# Autodesk Inventor assembly: 2016_IEEE_SouteastCon_Court
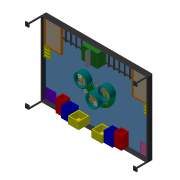
[picture p0: Inventor's stored thumbnail of the model, 180x180]
Saved by Autodesk Inventor 2015 (Build 190159000, 159)
## iProperties
Created: 2015-03-03
Part Number: 2016_IEEE_SouteastCon_Court
Document SubType Name: Assembly
Designer: Vukica
Author: Vukica
## Documents named in this file (16)
- C:\Users\Vukica\Dropbox\IEEE\hardware rules\2016Hardware_Court\2016_IEEE_SouteastCon_Court.iam
- C:\Users\Vukica\Dropbox\IEEE\hardware rules\2016Hardware_Court\Base.ipt
- C:\Users\Vukica\Dropbox\IEEE\hardware rules\2016Hardware_Court\Ship area.ipt
- C:\Users\Vukica\Dropbox\IEEE\hardware rules\2016Hardware_Court\Starting position pink.ipt
- C:\Users\Vukica\Dropbox\IEEE\hardware rules\2016Hardware_Court\Starting position purple.ipt
- C:\Users\Vukica\Dropbox\IEEE\hardware rules\2016Hardware_Court\Rail zone.ipt
- C:\Users\Vukica\Dropbox\IEEE\hardware rules\2016Hardware_Court\Beacon.ipt
- C:\Users\Vukica\Dropbox\IEEE\hardware rules\2016Hardware_Court\Side 84 in by 6 in by half inch.ipt
- C:\Users\Vukica\Dropbox\IEEE\hardware rules\2016Hardware_Court\Side 120 in by 6 in by half inch.ipt
- C:\Users\Vukica\Dropbox\IEEE\hardware rules\2016Hardware_Court\Hill.ipt
- C:\Users\Vukica\Dropbox\IEEE\hardware rules\2016Hardware_Court\Red truck.ipt
- C:\Users\Vukica\Dropbox\IEEE\hardware rules\2016Hardware_Court\Blue truck.ipt
- C:\Users\Vukica\Dropbox\IEEE\hardware rules\2016Hardware_Court\Yellow truck.ipt
- C:\Users\Vukica\Dropbox\IEEE\hardware rules\2016Hardware_Court\Island.ipt
- C:\Users\Vukica\Dropbox\IEEE\hardware rules\2016Hardware_Court\Gold bar.ipt
- C:\Users\Vukica\Dropbox\IEEE\hardware rules\2016Hardware_Court\White shipping good.ipt
## Components (43 placed, 15 different names)
1. Base:1 — Mate:1, Flush:1, Flush:2, Mate:2, Flush:3, Flush:4, Mate:3, Flush:5, Flush:6, Mate:4, Flush:7, Flush:8, Mate:5, Flush:9, Mate:7, Flush:11, Mate:9, Flush:12, Flush:13, Flush:15, Mate:10, Mate:11, Flush:16, Flush:18, Mate:12, Mate:17, Mate:20, Mate:22, Mate:25, Mate:28, Mate:30, Mate:33, Mate:36, Mate:38, Mate:40, Mate:43, Mate:46, Mate:53, Mate:55
2. Ship area:1 — Mate:1, Flush:1, Flush:2, Mate:6, Mate:49
3. Ship area:2 — Mate:2, Flush:3, Flush:4, Mate:8, Flush:10, Mate:54
4. Starting position pink:1 — Mate:4, Flush:7, Flush:8
5. Starting position purple:1 — Mate:3, Flush:5, Flush:6
6. Rail zone:1 — Mate:5, Mate:6, Flush:9
7. Rail zone:2 — Mate:7, Mate:8, Flush:10, Mate:18
8. Beacon:1 — Mate:14, Flush:22, Flush:23
9. Beacon:2 — Mate:13, Flush:20, Flush:21
10. Beacon:3 — Mate:15, Flush:24, Flush:25
11. Beacon:4 — Mate:16, Flush:26, Flush:27
12. Side 84 in by 6 in by half inch:1 — Mate:11, Flush:16, Flush:17, Mate:15, Flush:25, Mate:16, Flush:26, Flush:27
13. Side 84 in by 6 in by half inch:2 — Flush:18, Mate:12, Flush:19, Mate:13, Flush:21, Mate:14, Flush:23, Flush:28, Flush:29, Mate:39, Mate:41, Mate:44, Mate:47
14. Side 120 in by 6 in by half inch:1 — Flush:13, Flush:15, Mate:10, Flush:17, Flush:22, Flush:24, Mate:19, Mate:37
15. Side 120 in by 6 in by half inch:2 — Flush:11, Mate:9, Flush:12, Flush:19, Flush:20, Mate:21, Mate:23, Mate:26, Mate:29, Mate:32, Mate:34
16. Hill:1 — Mate:17, Mate:18, Mate:19
17. Red truck:1 — Mate:20, Mate:21, Flush:28, Mate:24
18. Blue truck:1 — Mate:22, Mate:23, Mate:24, Mate:27
19. Yellow truck:1 — Mate:25, Mate:26, Mate:27
20. Yellow truck:2 — Mate:33, Mate:34, Mate:35
21. Red truck:2 — Mate:28, Mate:29, Mate:31
22. Blue truck:2 — Mate:30, Mate:31, Mate:32, Mate:35
23. Island:1 — Mate:36, Flush:29, Mate:37
24. Gold bar:1 — Mate:38, Mate:39, Mate:42, Mate:45
25. Gold bar:2 — Mate:40, Mate:41, Mate:42, Mate:49
26. Gold bar:3 — Mate:43, Mate:44, Mate:45, Mate:48
27. Gold bar:4 — Mate:46, Mate:47, Mate:48
28. Gold bar:5 — Flush:30, Mate:50, Flush:31, Mate:51, Flush:32, Flush:33, Mate:53
29. Gold bar:6 — Flush:30, Mate:50, Flush:31, Mate:54, Mate:55
30. Gold bar:7 — Mate:51, Flush:32, Flush:33, Flush:34, Mate:52, Flush:35
31. Gold bar:8 — Flush:34, Mate:52, Flush:35
32. White shipping good:1
33. White shipping good:2
34. White shipping good:3
35. White shipping good:4
36. White shipping good:5
37. White shipping good:6
38. White shipping good:7
39. White shipping good:8
40. White shipping good:9
41. White shipping good:10
42. White shipping good:11
43. White shipping good:12
## Relationships (89: Mate 55, Flush 34)
- Mate:1: Base:1 ↔ Ship area:1
- Flush:1: Base:1 ↔ Ship area:1
- Flush:2: Base:1 ↔ Ship area:1
- Mate:2: Base:1 ↔ Ship area:2
- Flush:3: Base:1 ↔ Ship area:2
- Flush:4: Base:1 ↔ Ship area:2
- Mate:3: Base:1 ↔ Starting position purple:1
- Flush:5: Base:1 ↔ Starting position purple:1
- Flush:6: Base:1 ↔ Starting position purple:1
- Mate:4: Base:1 ↔ Starting position pink:1
- Flush:7: Base:1 ↔ Starting position pink:1
- Flush:8: Base:1 ↔ Starting position pink:1
- Mate:5: Base:1 ↔ Rail zone:1
- Mate:6: Ship area:1 ↔ Rail zone:1
- Flush:9: Base:1 ↔ Rail zone:1
- Mate:7: Base:1 ↔ Rail zone:2
- Mate:8: Ship area:2 ↔ Rail zone:2
- Flush:10: Ship area:2 ↔ Rail zone:2
- Flush:11: Base:1 ↔ Side 120 in by 6 in by half inch:2
- Mate:9: Base:1 ↔ Side 120 in by 6 in by half inch:2
- Flush:12: Base:1 ↔ Side 120 in by 6 in by half inch:2
- Flush:13: Base:1 ↔ Side 120 in by 6 in by half inch:1
- Flush:15: Base:1 ↔ Side 120 in by 6 in by half inch:1
- Mate:10: Base:1 ↔ Side 120 in by 6 in by half inch:1
- Mate:11: Base:1 ↔ Side 84 in by 6 in by half inch:1
- Flush:16: Base:1 ↔ Side 84 in by 6 in by half inch:1
- Flush:17: Side 84 in by 6 in by half inch:1 ↔ Side 120 in by 6 in by half inch:1
- Flush:18: Base:1 ↔ Side 84 in by 6 in by half inch:2
- Mate:12: Base:1 ↔ Side 84 in by 6 in by half inch:2
- Flush:19: Side 84 in by 6 in by half inch:2 ↔ Side 120 in by 6 in by half inch:2
- Mate:13: Beacon:2 ↔ Side 84 in by 6 in by half inch:2
- Flush:20: Beacon:2 ↔ Side 120 in by 6 in by half inch:2
- Flush:21: Beacon:2 ↔ Side 84 in by 6 in by half inch:2
- Mate:14: Beacon:1 ↔ Side 84 in by 6 in by half inch:2
- Flush:22: Beacon:1 ↔ Side 120 in by 6 in by half inch:1
- Flush:23: Beacon:1 ↔ Side 84 in by 6 in by half inch:2
- Mate:15: Beacon:3 ↔ Side 84 in by 6 in by half inch:1
- Flush:24: Beacon:3 ↔ Side 120 in by 6 in by half inch:1
- Flush:25: Beacon:3 ↔ Side 84 in by 6 in by half inch:1
- Mate:16: Beacon:4 ↔ Side 84 in by 6 in by half inch:1
- Flush:26: Beacon:4 ↔ Side 84 in by 6 in by half inch:1
- Flush:27: Beacon:4 ↔ Side 84 in by 6 in by half inch:1
- Mate:17: Base:1 ↔ Hill:1
- Mate:18: Rail zone:2 ↔ Hill:1
- Mate:19: Side 120 in by 6 in by half inch:1 ↔ Hill:1
- Mate:20: Base:1 ↔ Red truck:1
- Mate:21: Side 120 in by 6 in by half inch:2 ↔ Red truck:1
- Flush:28 (508 mm): Side 84 in by 6 in by half inch:2 ↔ Red truck:1
- Mate:22: Base:1 ↔ Blue truck:1
- Mate:23: Side 120 in by 6 in by half inch:2 ↔ Blue truck:1
- Mate:24: Red truck:1 ↔ Blue truck:1
- Mate:25: Base:1 ↔ Yellow truck:1
- Mate:26: Side 120 in by 6 in by half inch:2 ↔ Yellow truck:1
- Mate:27: Blue truck:1 ↔ Yellow truck:1
- Mate:28: Base:1 ↔ Red truck:2
- Mate:29: Side 120 in by 6 in by half inch:2 ↔ Red truck:2
- Mate:30: Base:1 ↔ Blue truck:2
- Mate:31: Red truck:2 ↔ Blue truck:2
- Mate:32: Side 120 in by 6 in by half inch:2 ↔ Blue truck:2
- Mate:33: Base:1 ↔ Yellow truck:2
- Mate:34: Side 120 in by 6 in by half inch:2 ↔ Yellow truck:2
- Mate:35: Yellow truck:2 ↔ Blue truck:2
- Mate:36: Base:1 ↔ Island:1
- Flush:29 (1524 mm): Side 84 in by 6 in by half inch:2 ↔ Island:1
- Mate:37 (-1016 mm): Side 120 in by 6 in by half inch:1 ↔ Island:1
- Mate:38: Base:1 ↔ Gold bar:1
- Mate:39: Side 84 in by 6 in by half inch:2 ↔ Gold bar:1
- Mate:40: Base:1 ↔ Gold bar:2
- Mate:41: Side 84 in by 6 in by half inch:2 ↔ Gold bar:2
- Mate:42: Gold bar:1 ↔ Gold bar:2
- Mate:43: Base:1 ↔ Gold bar:3
- Mate:44: Side 84 in by 6 in by half inch:2 ↔ Gold bar:3
- Mate:45: Gold bar:1 ↔ Gold bar:3
- Mate:46: Base:1 ↔ Gold bar:4
- Mate:47: Side 84 in by 6 in by half inch:2 ↔ Gold bar:4
- Mate:48: Gold bar:3 ↔ Gold bar:4
- Mate:49: Ship area:1 ↔ Gold bar:2
- Flush:30: Gold bar:5 ↔ Gold bar:6
- Mate:50: Gold bar:5 ↔ Gold bar:6
- Flush:31: Gold bar:5 ↔ Gold bar:6
- Mate:51: Gold bar:5 ↔ Gold bar:7
- Flush:32: Gold bar:5 ↔ Gold bar:7
- Flush:33: Gold bar:5 ↔ Gold bar:7
- Flush:34: Gold bar:7 ↔ Gold bar:8
- Mate:52: Gold bar:7 ↔ Gold bar:8
- Flush:35: Gold bar:7 ↔ Gold bar:8
- Mate:53: Base:1 ↔ Gold bar:5
- Mate:54: Ship area:2 ↔ Gold bar:6
- Mate:55: Base:1 ↔ Gold bar:6
